# Autodesk Inventor assembly: v1_Assembly1
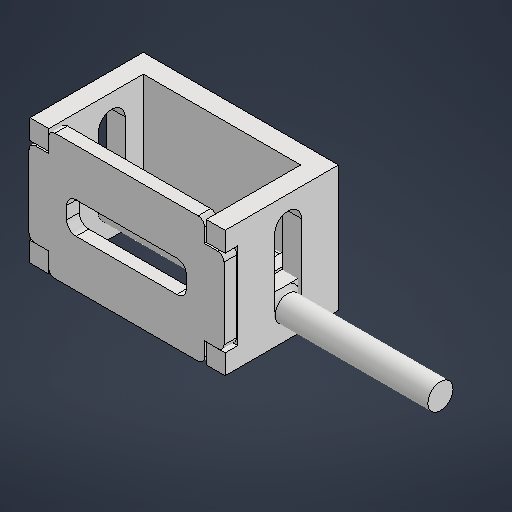
[picture p0: Inventor's stored thumbnail of the model, 512x512]
Saved by Autodesk Inventor 2026 (Build 300175050, 175E)
## iProperties
Created: 2025-09-02
Part Number: v1_Assembly1
Document SubType Name: Assembly
Designer: ka0n7
Author: ka0n7
## Documents named in this file (5)
- C:\Robohan\inventor2026\LRA Devices\Ex\v1\v1_Assembly1.iam
- C:\Robohan\inventor2026\LRA Devices\Ex\v1\main.ipt
- C:\Robohan\inventor2026\LRA Devices\Ex\v1\slidev.ipt
- C:\Robohan\inventor2026\LRA Devices\Ex\v1\VLV101040A.ipt
- C:\Robohan\inventor2026\LRA Devices\Ex\v1\top.ipt
## Components (5 placed, 4 different names)
1. main:1 — 角度:3, メイト:3, メイト:4
2. slidev:1 — メイト:1, 角度:1, フラッシュ:1, フラッシュ:2, フラッシュ:3, フラッシュ:4
3. slidev:2 — メイト:2, 角度:2, フラッシュ:1, フラッシュ:2, 角度:3
4. VLV101040A:1 — メイト:1, 角度:1, メイト:2, 角度:2, フラッシュ:3, フラッシュ:4
5. top:1 — メイト:3, メイト:4
## Relationships (11: Mate 4, Flush 4, Angle 3)
- メイト:1 [Mate]: slidev:1 ↔ VLV101040A:1
- 角度:1 [Angle] (0 deg): slidev:1 ↔ VLV101040A:1
- メイト:2 [Mate]: slidev:2 ↔ VLV101040A:1
- 角度:2 [Angle] (0 deg): slidev:2 ↔ VLV101040A:1
- フラッシュ:1 [Flush]: slidev:1 ↔ slidev:2
- フラッシュ:2 [Flush]: slidev:1 ↔ slidev:2
- フラッシュ:3 [Flush]: slidev:1 ↔ VLV101040A:1
- フラッシュ:4 [Flush] (-0.698 mm): slidev:1 ↔ VLV101040A:1
- 角度:3 [Angle] (0 deg): main:1 ↔ slidev:2
- メイト:3 [Mate]: main:1 ↔ top:1
- メイト:4 [Mate]: main:1 ↔ top:1
